# Autodesk Inventor assembly: BG201_trajan20_21
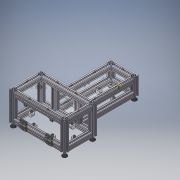
[picture p0: Inventor's stored thumbnail of the model, 180x180]
Saved by Autodesk Inventor 2022.2 (Build 262287000, 287)
## iProperties
Company: HTBLA Kaindorf
RuleStatus: InUse
Created: 2022-08-22
Part Number: BG201_trajan20_21
Project: Zeichenmaschine_v2
Material: Generisch
Description: gerüst_mit_platten
Document SubType Name: Assembly
Designer: trajan20
AfterDocNew0: iProperties-Editor_aufrufen
Author: jan
Keywords: 2021
## Documents named in this file (8)
- C:\Users\jan\Documents\DrawMachine\DrawMachineConstruction\Projekt\Zeichenmaschine_v2\BG201_trajan20_21_Zeichenmaschine_v2_gerüst_mit_platten.iam
- C:\Users\jan\Documents\DrawMachine\DrawMachineConstruction\Projekt\Zeichenmaschine_v2\BG103_trajan20_21_Zeichenmaschine_v2_Gerüst_Step_zu_Bauteil.iam
- C:\Users\jan\Documents\DrawMachine\DrawMachineConstruction\Projekt\Zeichenmaschine_v2\BT201_trajan20_21_Zeichenmaschine_v2_Hauptplatte unten.ipt
- C:\Users\jan\Documents\DrawMachine\DrawMachineConstruction\Projekt\Zeichenmaschine_v2\BT202_trajan20_21_Zeichenmaschine_v2_getriebemotor platte unten.ipt
- C:\Users\jan\Documents\DrawMachine\DrawMachineConstruction\Projekt\Zeichenmaschine_v2\BT101_trajan20_21_Zeichenmaschine_v2_Platte Stepper Motoren.ipt
- C:\Users\jan\Documents\DrawMachine\DrawMachineConstruction\Projekt\Zeichenmaschine_v2\BT102_trajan20_21_Zeichenmaschine_v2_Platte Getriebemotor.ipt
- C:\Users\jan\Documents\DrawMachine\DrawMachineConstruction\Projekt\Zeichenmaschine_v2\Normteile\de-DE\ISO 14583\ISO 14583 - M4x12-A3-70.ipt
- C:\Users\jan\Documents\DrawMachine\DrawMachineConstruction\Projekt\Zeichenmaschine_v2\DIN 7991 - M4x12_tx.ipt
## Components (17 placed, 7 different names)
1. BG103_trajan20_21_Zeichenmaschine_v2_Gerüst_Step_zu_Bauteil:1 [sub-assembly] — Passend:1, Passend:2, Passend:3, Passend:4, Passend:5, Passend:6, Passend:7, Fluchtend:1, Fluchtend:2, Fluchtend:3, Passend:8, Fluchtend:4
2. BT201_trajan20_21_Zeichenmaschine_v2_Hauptplatte unten:1 — Passend:1, Passend:2, Passend:3, Einfügen:1, Passend:9, Passend:10, Passend:11, Passend:12, Passend:13, Passend:14, Passend:15, Passend:16, Passend:17, Passend:18
3. BT202_trajan20_21_Zeichenmaschine_v2_getriebemotor platte unten:1 — Passend:4, Passend:5, Passend:6, Passend:19, Passend:20, Passend:21, Passend:22, Passend:23, Passend:24, Passend:25, Passend:26, Passend:27, Passend:28
4. BT101_trajan20_21_Zeichenmaschine_v2_Platte Stepper Motoren:1 — Passend:7, Fluchtend:1, Fluchtend:2
5. BT102_trajan20_21_Zeichenmaschine_v2_Platte Getriebemotor:1 — Fluchtend:3, Passend:8, Fluchtend:4
6. DIN 7991 M4x12:1
7. Schraube ISO 14583:2011(E) M4x12-A3-70:1 — Einfügen:1
8. Schraube ISO 14583:2011(E) M4x12-A3-70:2 — Passend:9, Passend:10
9. Schraube ISO 14583:2011(E) M4x12-A3-70:3 — Passend:11, Passend:12
10. Schraube ISO 14583:2011(E) M4x12-A3-70:4 — Passend:13, Passend:14
11. Schraube ISO 14583:2011(E) M4x12-A3-70:5 — Passend:15, Passend:16
12. Schraube ISO 14583:2011(E) M4x12-A3-70:6 — Passend:17, Passend:18
13. Schraube ISO 14583:2011(E) M4x12-A3-70:7 — Passend:19, Passend:20
14. Schraube ISO 14583:2011(E) M4x12-A3-70:8 — Passend:21, Passend:22
15. Schraube ISO 14583:2011(E) M4x12-A3-70:9 — Passend:23, Passend:24
16. Schraube ISO 14583:2011(E) M4x12-A3-70:10 — Passend:25, Passend:26
17. Schraube ISO 14583:2011(E) M4x12-A3-70:11 — Passend:27, Passend:28
## Relationships (33: Mate 28, Flush 4, Insert 1)
- Passend:1 [Mate]: BG103_trajan20_21_Zeichenmaschine_v2_Gerüst_Step_zu_Bauteil:1 ↔ BT201_trajan20_21_Zeichenmaschine_v2_Hauptplatte unten:1
- Passend:2 [Mate]: BG103_trajan20_21_Zeichenmaschine_v2_Gerüst_Step_zu_Bauteil:1 ↔ BT201_trajan20_21_Zeichenmaschine_v2_Hauptplatte unten:1
- Passend:3 [Mate]: BG103_trajan20_21_Zeichenmaschine_v2_Gerüst_Step_zu_Bauteil:1 ↔ BT201_trajan20_21_Zeichenmaschine_v2_Hauptplatte unten:1
- Passend:4 [Mate]: BG103_trajan20_21_Zeichenmaschine_v2_Gerüst_Step_zu_Bauteil:1 ↔ BT202_trajan20_21_Zeichenmaschine_v2_getriebemotor platte unten:1
- Passend:5 [Mate]: BG103_trajan20_21_Zeichenmaschine_v2_Gerüst_Step_zu_Bauteil:1 ↔ BT202_trajan20_21_Zeichenmaschine_v2_getriebemotor platte unten:1
- Passend:6 [Mate]: BG103_trajan20_21_Zeichenmaschine_v2_Gerüst_Step_zu_Bauteil:1 ↔ BT202_trajan20_21_Zeichenmaschine_v2_getriebemotor platte unten:1
- Passend:7 [Mate]: BG103_trajan20_21_Zeichenmaschine_v2_Gerüst_Step_zu_Bauteil:1 ↔ BT101_trajan20_21_Zeichenmaschine_v2_Platte Stepper Motoren:1
- Fluchtend:1 [Flush]: BG103_trajan20_21_Zeichenmaschine_v2_Gerüst_Step_zu_Bauteil:1 ↔ BT101_trajan20_21_Zeichenmaschine_v2_Platte Stepper Motoren:1
- Fluchtend:2 [Flush]: BG103_trajan20_21_Zeichenmaschine_v2_Gerüst_Step_zu_Bauteil:1 ↔ BT101_trajan20_21_Zeichenmaschine_v2_Platte Stepper Motoren:1
- Fluchtend:3 [Flush]: BG103_trajan20_21_Zeichenmaschine_v2_Gerüst_Step_zu_Bauteil:1 ↔ BT102_trajan20_21_Zeichenmaschine_v2_Platte Getriebemotor:1
- Passend:8 [Mate]: BG103_trajan20_21_Zeichenmaschine_v2_Gerüst_Step_zu_Bauteil:1 ↔ BT102_trajan20_21_Zeichenmaschine_v2_Platte Getriebemotor:1
- Fluchtend:4 [Flush]: BG103_trajan20_21_Zeichenmaschine_v2_Gerüst_Step_zu_Bauteil:1 ↔ BT102_trajan20_21_Zeichenmaschine_v2_Platte Getriebemotor:1
- Einfügen:1 [Insert]: BT201_trajan20_21_Zeichenmaschine_v2_Hauptplatte unten:1 ↔ Schraube ISO 14583:2011(E) M4x12-A3-70:1
- Passend:9 [Mate]: BT201_trajan20_21_Zeichenmaschine_v2_Hauptplatte unten:1 ↔ Schraube ISO 14583:2011(E) M4x12-A3-70:2
- Passend:10 [Mate]: BT201_trajan20_21_Zeichenmaschine_v2_Hauptplatte unten:1 ↔ Schraube ISO 14583:2011(E) M4x12-A3-70:2
- Passend:11 [Mate]: BT201_trajan20_21_Zeichenmaschine_v2_Hauptplatte unten:1 ↔ Schraube ISO 14583:2011(E) M4x12-A3-70:3
- Passend:12 [Mate]: BT201_trajan20_21_Zeichenmaschine_v2_Hauptplatte unten:1 ↔ Schraube ISO 14583:2011(E) M4x12-A3-70:3
- Passend:13 [Mate]: BT201_trajan20_21_Zeichenmaschine_v2_Hauptplatte unten:1 ↔ Schraube ISO 14583:2011(E) M4x12-A3-70:4
- Passend:14 [Mate]: BT201_trajan20_21_Zeichenmaschine_v2_Hauptplatte unten:1 ↔ Schraube ISO 14583:2011(E) M4x12-A3-70:4
- Passend:15 [Mate]: BT201_trajan20_21_Zeichenmaschine_v2_Hauptplatte unten:1 ↔ Schraube ISO 14583:2011(E) M4x12-A3-70:5
- Passend:16 [Mate]: BT201_trajan20_21_Zeichenmaschine_v2_Hauptplatte unten:1 ↔ Schraube ISO 14583:2011(E) M4x12-A3-70:5
- Passend:17 [Mate]: BT201_trajan20_21_Zeichenmaschine_v2_Hauptplatte unten:1 ↔ Schraube ISO 14583:2011(E) M4x12-A3-70:6
- Passend:18 [Mate]: BT201_trajan20_21_Zeichenmaschine_v2_Hauptplatte unten:1 ↔ Schraube ISO 14583:2011(E) M4x12-A3-70:6
- Passend:19 [Mate]: BT202_trajan20_21_Zeichenmaschine_v2_getriebemotor platte unten:1 ↔ Schraube ISO 14583:2011(E) M4x12-A3-70:7
- Passend:20 [Mate]: BT202_trajan20_21_Zeichenmaschine_v2_getriebemotor platte unten:1 ↔ Schraube ISO 14583:2011(E) M4x12-A3-70:7
- Passend:21 [Mate]: BT202_trajan20_21_Zeichenmaschine_v2_getriebemotor platte unten:1 ↔ Schraube ISO 14583:2011(E) M4x12-A3-70:8
- Passend:22 [Mate]: BT202_trajan20_21_Zeichenmaschine_v2_getriebemotor platte unten:1 ↔ Schraube ISO 14583:2011(E) M4x12-A3-70:8
- Passend:23 [Mate]: BT202_trajan20_21_Zeichenmaschine_v2_getriebemotor platte unten:1 ↔ Schraube ISO 14583:2011(E) M4x12-A3-70:9
- Passend:24 [Mate]: BT202_trajan20_21_Zeichenmaschine_v2_getriebemotor platte unten:1 ↔ Schraube ISO 14583:2011(E) M4x12-A3-70:9
- Passend:25 [Mate]: BT202_trajan20_21_Zeichenmaschine_v2_getriebemotor platte unten:1 ↔ Schraube ISO 14583:2011(E) M4x12-A3-70:10
- Passend:26 [Mate]: BT202_trajan20_21_Zeichenmaschine_v2_getriebemotor platte unten:1 ↔ Schraube ISO 14583:2011(E) M4x12-A3-70:10
- Passend:27 [Mate]: BT202_trajan20_21_Zeichenmaschine_v2_getriebemotor platte unten:1 ↔ Schraube ISO 14583:2011(E) M4x12-A3-70:11
- Passend:28 [Mate]: BT202_trajan20_21_Zeichenmaschine_v2_getriebemotor platte unten:1 ↔ Schraube ISO 14583:2011(E) M4x12-A3-70:11
